# Autodesk Inventor assembly: MotorBlock
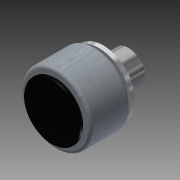
[picture p0: Inventor's stored thumbnail of the model, 180x180]
Saved by Autodesk Inventor 2014 SP1 (Build 180222100, 222)
## iProperties
Created: 2015-03-22
Part Number: MotorBlock
Document SubType Name: Assembly
Designer: david
Mass: 165.571 g
Surface Area: 186.805 cm^2
Volume: 59.5858 cm^3
Density: 2.7787 g/cm^3
Author: david
## Documents named in this file (3)
- C:\Users\asus\Documents\Autodesk\Projects\AUSBEEDone\Components\MotorBlock.iam
- C:\Users\asus\Documents\Autodesk\Projects\AUSBEEDone\Components\Motor.ipt
- C:\Users\asus\Documents\Autodesk\Projects\AUSBEEDone\Components\MotorWheel.ipt
## Components (2 placed, 2 different names)
1. Motor:1 — Tangent:1, Mate:1
2. MotorWheel:1 — Tangent:1, Mate:1
## Relationships (2: Tangent 1, Mate 1)
- Tangent:1: Motor:1 ↔ MotorWheel:1
- Mate:1: Motor:1 ↔ MotorWheel:1
